# Autodesk Inventor assembly: Thorax
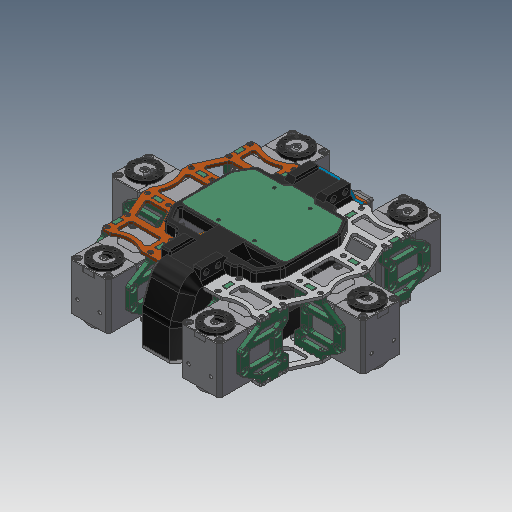
[picture p0: Inventor's stored thumbnail of the model, 512x512]
Saved by Autodesk Inventor 2019.4 (Build 234330000, 330)
## iProperties
Created: 2018-08-06
Part Number: Thorax
Material: 一般
Document SubType Name: Assembly
Designer: student
Author: student
## Documents named in this file (12)
- C:\Workspace\Yunit8-HaptHexa\Hardware\Inventor\Thorax\_Thorax.iam
- C:\Workspace\Yunit8-HaptHexa\Hardware\Inventor\Thorax\yaw_unit\yaw_unit.iam
- C:\Workspace\Yunit8-HaptHexa\Hardware\Inventor\Thorax\kypom_3s_2500.ipt
- C:\Workspace\Yunit8-HaptHexa\Hardware\Inventor\Thorax\U2D2.ipt
- C:\Workspace\Yunit8-HaptHexa\Hardware\Inventor\Thorax\body_bottom.ipt
- C:\Workspace\Yunit8-HaptHexa\Hardware\Inventor\Thorax\body_top.ipt
- C:\Workspace\Yunit8-HaptHexa\Hardware\Inventor\Thorax\battery_cover_v2.ipt
- C:\Workspace\Yunit8-HaptHexa\Hardware\Inventor\Thorax\battery_holder_back.ipt
- C:\Workspace\Yunit8-HaptHexa\Hardware\Inventor\Thorax\battery_lib_assy.iam
- C:\Workspace\Yunit8-HaptHexa\Hardware\Inventor\Thorax\body_top_mir.ipt
- C:\Workspace\Yunit8-HaptHexa\Hardware\Inventor\Thorax\main_pcb.ipt
- C:\Workspace\Yunit8-HaptHexa\Hardware\Inventor\Thorax\yaw_unit\yaw_unit_mir1.iam
## Components (15 placed, 11 different names)
1. battery_cover_v2:1 — フラッシュ:1, フラッシュ:2, フラッシュ:3, メイト:46, メイト:47, メイト:48, メイト:49, メイト:50
2. kypom_3s_2500:1
3. U2D2:1 — メイト:45, メイト:46, メイト:48
4. body_bottom:1 — メイト:4, メイト:5, メイト:17, メイト:18, メイト:23, メイト:24, メイト:26, メイト:27, フラッシュ:51, フラッシュ:52, フラッシュ:53, メイト:49
5. battery_holder_back:1 — メイト:20, フラッシュ:5, メイト:34, メイト:35, メイト:50, メイト:51
6. battery_lib_assy:1 [sub-assembly] — メイト:34, メイト:35, メイト:51
7. body_top:1 — メイト:42, メイト:43, フラッシュ:6
8. body_top_mir:1
9. main_pcb:1 — メイト:47, フラッシュ:49, フラッシュ:50
10. yaw_unit:1 [sub-assembly] — メイト:26, メイト:27, フラッシュ:51
11. yaw_unit:2 [sub-assembly] — メイト:23, メイト:24, メイト:42, メイト:43, フラッシュ:6, フラッシュ:52
12. yaw_unit:3 [sub-assembly] — メイト:17, メイト:18, メイト:45, フラッシュ:53
13. yaw_unit_mir1:1 [sub-assembly]
14. yaw_unit_mir1:2 [sub-assembly]
15. yaw_unit_mir1:3 [sub-assembly]
## Relationships (30: Mate 20, Flush 10)
- メイト:4 [Mate]: body_bottom:1
- メイト:5 [Mate]: body_bottom:1
- フラッシュ:1 [Flush]: battery_cover_v2:1
- フラッシュ:2 [Flush]: battery_cover_v2:1
- フラッシュ:3 [Flush]: battery_cover_v2:1
- メイト:17 [Mate]: body_bottom:1 ↔ yaw_unit:3
- メイト:18 [Mate]: body_bottom:1 ↔ yaw_unit:3
- メイト:20 [Mate]: battery_holder_back:1
- フラッシュ:5 [Flush]: battery_holder_back:1
- メイト:23 [Mate]: body_bottom:1 ↔ yaw_unit:2
- メイト:24 [Mate]: body_bottom:1 ↔ yaw_unit:2
- メイト:26 [Mate]: body_bottom:1 ↔ yaw_unit:1
- メイト:27 [Mate]: body_bottom:1 ↔ yaw_unit:1
- メイト:34 [Mate]: battery_holder_back:1 ↔ battery_lib_assy:1
- メイト:35 [Mate]: battery_holder_back:1 ↔ battery_lib_assy:1
- メイト:42 [Mate]: body_top:1 ↔ yaw_unit:2
- メイト:43 [Mate]: body_top:1 ↔ yaw_unit:2
- フラッシュ:6 [Flush]: body_top:1 ↔ yaw_unit:2
- メイト:45 [Mate] (2 mm): U2D2:1 ↔ yaw_unit:3
- メイト:46 [Mate] (3 mm): battery_cover_v2:1 ↔ U2D2:1
- メイト:47 [Mate]: battery_cover_v2:1 ↔ main_pcb:1
- フラッシュ:49 [Flush]: main_pcb:1
- フラッシュ:50 [Flush]: main_pcb:1
- メイト:48 [Mate]: battery_cover_v2:1 ↔ U2D2:1
- フラッシュ:51 [Flush]: body_bottom:1 ↔ yaw_unit:1
- フラッシュ:52 [Flush]: body_bottom:1 ↔ yaw_unit:2
- フラッシュ:53 [Flush]: body_bottom:1 ↔ yaw_unit:3
- メイト:49 [Mate]: battery_cover_v2:1 ↔ body_bottom:1
- メイト:50 [Mate]: battery_cover_v2:1 ↔ battery_holder_back:1
- メイト:51 [Mate]: battery_holder_back:1 ↔ battery_lib_assy:1
